# Autodesk Inventor assembly: aa FINAL MODEL with drainage extension
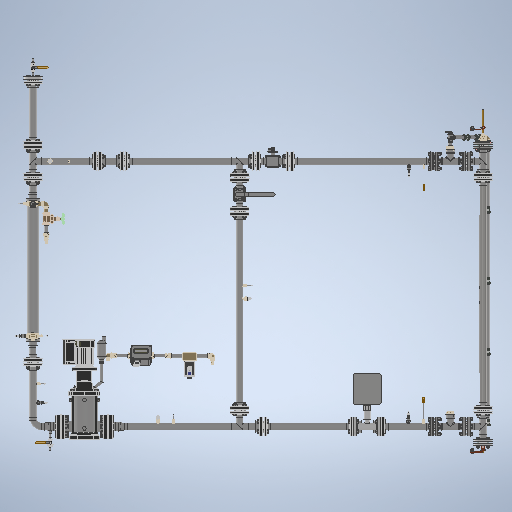
[picture p0: Inventor's stored thumbnail of the model, 512x512]
Saved by Autodesk Inventor 2027 (Build 310192000, 192)
## iProperties
Created: 2026-07-30
Part Number: aa FINAL MODEL with drainage extension
Document SubType Name: Assembly
Designer: AdminForWorker
Title: aa FINAL MODEL with drainage extension v22
Author: AdminForWorker
## Documents named in this file (45)
- C:\Users\ig2\Desktop\SMR Thermal\thermal-loop\resources\v0.1.2\CAD\Inventor\aa FINAL MODEL with proportional valve\aa FINAL MODEL with drainage extension.iam
- C:\Users\ig2\Desktop\SMR Thermal\thermal-loop\resources\v0.1.2\CAD\Inventor\aa FINAL MODEL with proportional valve\Average Flange Component (Larger Nut) v13.iam
- C:\Users\ig2\Desktop\SMR Thermal\thermal-loop\resources\v0.1.2\CAD\Inventor\aa FINAL MODEL with proportional valve\Average Flange Component (Larger Nut) v13_1.iam
- C:\Users\ig2\Desktop\SMR Thermal\thermal-loop\resources\v0.1.2\CAD\Inventor\aa FINAL MODEL with proportional valve\Flow-Tek Large Valve v6.ipt
- C:\Users\ig2\Desktop\SMR Thermal\thermal-loop\resources\v0.1.2\CAD\Inventor\aa FINAL MODEL with proportional valve\Average Flange Component (Larger Nut) v13_2.iam
- C:\Users\ig2\Desktop\SMR Thermal\thermal-loop\resources\v0.1.2\CAD\Inventor\aa FINAL MODEL with proportional valve\T pipe v3.ipt
- C:\Users\ig2\Desktop\SMR Thermal\thermal-loop\resources\v0.1.2\CAD\Inventor\aa FINAL MODEL with proportional valve\Average Flange Component (Larger Nut) v13_3.iam
- C:\Users\ig2\Desktop\SMR Thermal\thermal-loop\resources\v0.1.2\CAD\Inventor\aa FINAL MODEL with proportional valve\Average Flange Component (Larger Nut) v13_4.iam
- C:\Users\ig2\Desktop\SMR Thermal\thermal-loop\resources\v0.1.2\CAD\Inventor\aa FINAL MODEL with proportional valve\MC-II Flow Analyzer v7.iam
- C:\Users\ig2\Desktop\SMR Thermal\thermal-loop\resources\v0.1.2\CAD\Inventor\aa FINAL MODEL with proportional valve\Small I pipe v2.ipt
- C:\Users\ig2\Desktop\SMR Thermal\thermal-loop\resources\v0.1.2\CAD\Inventor\aa FINAL MODEL with proportional valve\Average Flange Component (Smaller Nut) v7.iam
- C:\Users\ig2\Desktop\SMR Thermal\thermal-loop\resources\v0.1.2\CAD\Inventor\aa FINAL MODEL with proportional valve\Pipe II v3.ipt
- C:\Users\ig2\Desktop\SMR Thermal\thermal-loop\resources\v0.1.2\CAD\Inventor\aa FINAL MODEL with proportional valve\Heater Connection Flange w_ rod v8.iam
- C:\Users\ig2\Desktop\SMR Thermal\thermal-loop\resources\v0.1.2\CAD\Inventor\aa FINAL MODEL with proportional valve\regular pipe to pump pipe connector v3.ipt
- C:\Users\ig2\Desktop\SMR Thermal\thermal-loop\resources\v0.1.2\CAD\Inventor\aa FINAL MODEL with proportional valve\Large Pump Flange v5.iam
- C:\Users\ig2\Desktop\SMR Thermal\thermal-loop\resources\v0.1.2\CAD\Inventor\aa FINAL MODEL with proportional valve\pump v5.iam
- C:\Users\ig2\Desktop\SMR Thermal\thermal-loop\resources\v0.1.2\CAD\Inventor\aa FINAL MODEL with proportional valve\Large Pump Flange v5_1.iam
- C:\Users\ig2\Desktop\SMR Thermal\thermal-loop\resources\v0.1.2\CAD\Inventor\aa FINAL MODEL with proportional valve\Water Drainage Valve v5.iam
- C:\Users\ig2\Desktop\SMR Thermal\thermal-loop\resources\v0.1.2\CAD\Inventor\aa FINAL MODEL with proportional valve\Pipe D v2.ipt
- C:\Users\ig2\Desktop\SMR Thermal\thermal-loop\resources\v0.1.2\CAD\Inventor\aa FINAL MODEL with proportional valve\Average Flange Component (Larger Nut) v13_5.iam
- C:\Users\ig2\Desktop\SMR Thermal\thermal-loop\resources\v0.1.2\CAD\Inventor\aa FINAL MODEL with proportional valve\Pipe C v2.ipt
- C:\Users\ig2\Desktop\SMR Thermal\thermal-loop\resources\v0.1.2\CAD\Inventor\aa FINAL MODEL with proportional valve\Average Flange Component (Larger Nut) v13_6.iam
- C:\Users\ig2\Desktop\SMR Thermal\thermal-loop\resources\v0.1.2\CAD\Inventor\aa FINAL MODEL with proportional valve\elbow 90_ pipe v5.ipt
- C:\Users\ig2\Desktop\SMR Thermal\thermal-loop\resources\v0.1.2\CAD\Inventor\aa FINAL MODEL with proportional valve\Average Flange Component (Larger Nut) v13_7.iam
- C:\Users\ig2\Desktop\SMR Thermal\thermal-loop\resources\v0.1.2\CAD\Inventor\aa FINAL MODEL with proportional valve\Short Piece for Tube v2.ipt
- C:\Users\ig2\Desktop\SMR Thermal\thermal-loop\resources\v0.1.2\CAD\Inventor\aa FINAL MODEL with proportional valve\Average Flange Component (Larger Nut) v13_8.iam
- C:\Users\ig2\Desktop\SMR Thermal\thermal-loop\resources\v0.1.2\CAD\Inventor\aa FINAL MODEL with proportional valve\Average Flange Component (Larger Nut) v13_9.iam
- C:\Users\ig2\Desktop\SMR Thermal\thermal-loop\resources\v0.1.2\CAD\Inventor\aa FINAL MODEL with proportional valve\Pipe A v4.ipt
- C:\Users\ig2\Desktop\SMR Thermal\thermal-loop\resources\v0.1.2\CAD\Inventor\aa FINAL MODEL with proportional valve\Air Exhaust Valve v11.iam
- C:\Users\ig2\Desktop\SMR Thermal\thermal-loop\resources\v0.1.2\CAD\Inventor\aa FINAL MODEL with proportional valve\Welded Extension Section Final v5.iam
- C:\Users\ig2\Desktop\SMR Thermal\thermal-loop\resources\v0.1.2\CAD\Inventor\aa FINAL MODEL with proportional valve\Average Flange Component (Smaller Nut) v7_1.iam
- C:\Users\ig2\Desktop\SMR Thermal\thermal-loop\resources\v0.1.2\CAD\Inventor\aa FINAL MODEL with proportional valve\Average Flange Component (Smaller Nut) v7_2.iam
- C:\Users\ig2\Desktop\SMR Thermal\thermal-loop\resources\v0.1.2\CAD\Inventor\aa FINAL MODEL with proportional valve\PipeAssembly1 v4.iam
- C:\Users\ig2\Desktop\SMR Thermal\thermal-loop\resources\v0.1.2\CAD\Inventor\aa FINAL MODEL with proportional valve\Welded Extension Section w_ relief v10.iam
- C:\Users\ig2\Desktop\SMR Thermal\thermal-loop\resources\v0.1.2\CAD\Inventor\aa FINAL MODEL with proportional valve\Top right non pressure relief v13.iam
- C:\Users\ig2\Desktop\SMR Thermal\thermal-loop\resources\v0.1.2\CAD\Inventor\aa FINAL MODEL with proportional valve\Extension plug v3.ipt
- C:\Users\ig2\Desktop\SMR Thermal\thermal-loop\resources\v0.1.2\CAD\Inventor\aa FINAL MODEL with proportional valve\Pipe J w_ sensors v3.iam
- C:\Users\ig2\Desktop\SMR Thermal\thermal-loop\resources\v0.1.2\CAD\Inventor\aa FINAL MODEL with proportional valve\Pipe E w_ sensors v2.iam
- C:\Users\ig2\Desktop\SMR Thermal\thermal-loop\resources\v0.1.2\CAD\Inventor\aa FINAL MODEL with proportional valve\Pipe I w_ sensors v1.iam
- C:\Users\ig2\Desktop\SMR Thermal\thermal-loop\resources\v0.1.2\CAD\Inventor\aa FINAL MODEL with proportional valve\Pipe H w_ sensors v1.iam
- C:\Users\ig2\Desktop\SMR Thermal\thermal-loop\resources\v0.1.2\CAD\Inventor\aa FINAL MODEL with proportional valve\Pipe B w_ sensors v1.iam
- C:\Users\ig2\Desktop\SMR Thermal\thermal-loop\resources\v0.1.2\CAD\Inventor\aa FINAL MODEL with proportional valve\Pipe F w_ sensors v1.iam
- C:\Users\ig2\Desktop\SMR Thermal\thermal-loop\resources\v0.1.2\CAD\Inventor\aa FINAL MODEL with proportional valve\Heat Exchanger w_ parts v8.iam
- C:\Users\ig2\Desktop\SMR Thermal\thermal-loop\resources\v0.1.2\CAD\Inventor\aa FINAL MODEL with proportional valve\Proportional valve setup v1.iam
- C:\Users\ig2\Desktop\SMR Thermal\thermal-loop\resources\v0.1.2\CAD\Inventor\aa FINAL MODEL with proportional valve\switch pipe valve v2.ipt
## Components (50 placed, 32 different names)
1. Average Flange Component (Larger Nut) v13:1 [sub-assembly]
2. Average Flange Component (Larger Nut) v13:2 [sub-assembly]
3. Flow-Tek Large Valve v6:1
4. Average Flange Component (Larger Nut) v13:3 [sub-assembly]
5. T pipe v3:2
6. Average Flange Component (Larger Nut) v13:4 [sub-assembly]
7. Average Flange Component (Larger Nut) v13:5 [sub-assembly]
8. Flow-Tek Large Valve v6:2
9. T pipe v3:3
10. T pipe v3:4
11. T pipe v3:5
12. MC-II Flow Analyzer v7:1 [sub-assembly]
13. Small I pipe v2:1
14. Average Flange Component (Smaller Nut) v7:3 [sub-assembly]
15. Pipe II v3:1
16. Heater Connection Flange w/ rod v8:1 [sub-assembly]
17. regular pipe to pump pipe connector v3:1
18. Large Pump Flange v5:1 [sub-assembly]
19. pump v5:1 [sub-assembly]
20. Large Pump Flange v5:2 [sub-assembly]
21. Water Drainage Valve v5:1 [sub-assembly]
22. Pipe D v2:1
23. Average Flange Component (Larger Nut) v13:6 [sub-assembly]
24. Pipe C v2:1
25. Average Flange Component (Larger Nut) v13:7 [sub-assembly]
26. elbow 90* pipe v5:1
27. Average Flange Component (Larger Nut) v13:8 [sub-assembly]
28. Short Piece for Tube v2:1
29. Short Piece for Tube v2:2
30. Average Flange Component (Larger Nut) v13:9 [sub-assembly]
31. T pipe v3:6
32. Average Flange Component (Larger Nut) v13:10 [sub-assembly]
33. Pipe A v4:1
34. Air Exhaust Valve v11:1 [sub-assembly]
35. Welded Extension Section Final v5:2 [sub-assembly]
36. Average Flange Component (Smaller Nut) v7:4 [sub-assembly]
37. Average Flange Component (Smaller Nut) v7:5 [sub-assembly]
38. PipeAssembly1 v4:1 [sub-assembly]
39. Welded Extension Section w/ relief v10:1 [sub-assembly]
40. Top right non pressure relief v13:1 [sub-assembly]
41. Extension plug v3:1
42. Pipe J w/ sensors v3:1 [sub-assembly]
43. Pipe E w/ sensors v2:1 [sub-assembly]
44. Pipe I w/ sensors v1:1 [sub-assembly]
45. Pipe H w/ sensors v1:1 [sub-assembly]
46. Pipe B w/ sensors v1:1 [sub-assembly]
47. Pipe F w/ sensors v1:1 [sub-assembly]
48. Heat Exchanger w/ parts v8:1 [sub-assembly] — Rotational:1
49. Proportional valve setup v1:1 [sub-assembly]
50. switch pipe valve v2:1 — Rotational:1
## Relationships (1: RevoluteJoint 1)
- Rotational:1 [RevoluteJoint]: Heat Exchanger w/ parts v8:1 ↔ switch pipe valve v2:1
